# Autodesk Inventor assembly: Federundschraube_ra8846s
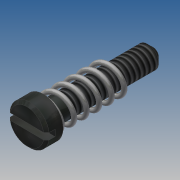
[picture p0: Inventor's stored thumbnail of the model, 180x180]
Saved by Autodesk Inventor 2021 (Build 250183000, 183)
## iProperties
Created: 2021-01-14
Part Number: Federundschraube_ra8846s
Document SubType Name: Assembly
Designer: Sander
Author: Sander
## Documents named in this file (4)
- C:\Users\ricar\OneDrive - Fachhochschule Aachen\Mechatronik I\CAD\INVENTOR\Proyectos\Daten\Federundschraube_ra8846s.iam
- C:\Users\ricar\OneDrive - Fachhochschule Aachen\Mechatronik I\CAD\INVENTOR\Proyectos\Daten\Feder_ra8846s.ipt
- C:\Users\ricar\OneDrive - Fachhochschule Aachen\Mechatronik I\CAD\INVENTOR\Proyectos\Daten\Schlitzschraube_ra8846s\Schlitzschraube_ra8846s-02.ipt
- C:\Users\ricar\OneDrive - Fachhochschule Aachen\Mechatronik I\CAD\INVENTOR\Proyectos\Daten\Schlitzschraube_ra8846s.ipt
## Components (2 placed, 2 different names)
1. Feder_ra8846s:1 — Passend:1, Tangential:1
2. Schlitzschraube_ra8846s-02:1 — Passend:1, Tangential:1
## Relationships (2: Mate 1, Tangent 1)
- Passend:1 [Mate]: Feder_ra8846s:1 ↔ Schlitzschraube_ra8846s-02:1
- Tangential:1: Feder_ra8846s:1 ↔ Schlitzschraube_ra8846s-02:1
